# Autodesk Inventor assembly: AVT-32-16
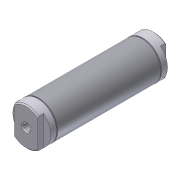
[picture p0: Inventor's stored thumbnail of the model, 180x180]
Saved by Autodesk Inventor 2013 (Build 170138000, 138)
## iProperties
Category: Pneumatics
Created: 2007-11-13
Part Number: AVT-32-16
Document SubType Name: Assembly
Catalog Web Link: http://www.clippard.com/store/display_details.asp?sku=AVT-32-16
Description: Accumulator
Vendor: Clippard
Mass: 615.197 g
Surface Area: 604.406 cm^2
Volume: 113.327 cm^3
Density: 5.4285 g/cm^3
Project: FIRST
Title: Accumulator
Author: Autodesk, Inc.
## Documents named in this file (3)
- C:\Users\Moses\Documents\GitHub\frc2013CAD\Pneumatics\Pneumatics_Clippard_AVT-32-16.iam
- C:\Users\Moses\Documents\GitHub\frc2013CAD\Pneumatics\AVT-32-16_Body Tube.ipt
- C:\Users\Moses\Documents\GitHub\frc2013CAD\Pneumatics\AVT-32-16_End Cap.ipt
## Components (3 placed, 2 different names)
1. AVT-32-16_Body Tube:1 — Insert:1, Insert:2, Angle:1, Angle:2
2. AVT-32-16_End Cap:1 — Insert:1, Angle:1
3. AVT-32-16_End Cap:2 — Insert:2, Angle:2
## Relationships (4: Insert 2, Angle 2)
- Insert:1: AVT-32-16_Body Tube:1 ↔ AVT-32-16_End Cap:1
- Insert:2: AVT-32-16_Body Tube:1 ↔ AVT-32-16_End Cap:2
- Angle:1 (0 deg): AVT-32-16_Body Tube:1 ↔ AVT-32-16_End Cap:1
- Angle:2 (0 deg): AVT-32-16_Body Tube:1 ↔ AVT-32-16_End Cap:2
